# Autodesk Inventor assembly: base_assembly
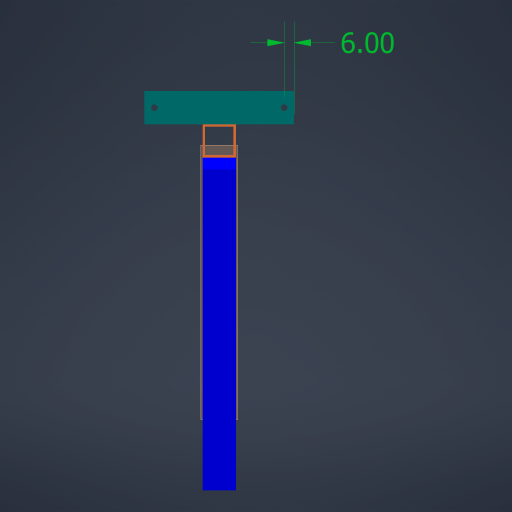
[picture p0: Inventor's stored thumbnail of the model, 512x512]
Saved by Autodesk Inventor 2024 (Build 280153000, 153)
## iProperties
Created: 2023-04-14
Part Number: base_assembly
Document SubType Name: Assembly
Designer: user
Author: user
## Documents named in this file (5)
- D:\Docs\Robot\3d\base\base_assembly.iam
- D:\Docs\Robot\3d\base\main axis.ipt
- D:\Docs\Robot\3d\base\section.ipt
- D:\Docs\Robot\3d\base\shock_absorber_holder_down_150.ipt
- D:\Docs\Robot\3d\base\shock_absorber_holder_down_200.ipt
## Components (8 placed, 4 different names)
1. main axis:1 — Совмещение:1, Совмещение:2, Плоский:1, Плоский:5, Плоский:6, Плоский:8, Совмещение:37, Совмещение:38, Совмещение:41, Совмещение:48, Совмещение:50, Совмещение:52
2. section:1 — Совмещение:1, Совмещение:2, Совмещение:46, Совмещение:49
3. section:3
4. section:4
5. section:5 — Совмещение:45, Совмещение:47, Совмещение:48, Совмещение:49
6. shock_absorber_holder_down_150:1 — Плоский:1, Плоский:8, Совмещение:37, Совмещение:52
7. shock_absorber_holder_down_150:2 — Плоский:5, Плоский:6, Совмещение:50, Совмещение:51
8. shock_absorber_holder_down_200:1 — Совмещение:38, Совмещение:41, Совмещение:51
## Relationships (17: Mate 13, PlanarJoint 4)
- Совмещение:1 [Mate]: main axis:1 ↔ section:1
- Совмещение:2 [Mate] (55 mm): main axis:1 ↔ section:1
- Плоский:1 [PlanarJoint]: main axis:1 ↔ shock_absorber_holder_down_150:1
- Плоский:5 [PlanarJoint]: main axis:1 ↔ shock_absorber_holder_down_150:2
- Плоский:6 [PlanarJoint]: main axis:1 ↔ shock_absorber_holder_down_150:2
- Плоский:8 [PlanarJoint]: main axis:1 ↔ shock_absorber_holder_down_150:1
- Совмещение:37 [Mate]: main axis:1 ↔ shock_absorber_holder_down_150:1
- Совмещение:38 [Mate]: main axis:1 ↔ shock_absorber_holder_down_200:1
- Совмещение:41 [Mate]: main axis:1 ↔ shock_absorber_holder_down_200:1
- Совмещение:45 [Mate]: section:5
- Совмещение:46 [Mate]: section:1
- Совмещение:47 [Mate]: section:5
- Совмещение:48 [Mate]: main axis:1 ↔ section:5
- Совмещение:49 [Mate]: section:1 ↔ section:5
- Совмещение:50 [Mate] (55 mm): main axis:1 ↔ shock_absorber_holder_down_150:2
- Совмещение:51 [Mate] (117 mm): shock_absorber_holder_down_150:2 ↔ shock_absorber_holder_down_200:1
- Совмещение:52 [Mate] (55 mm): main axis:1 ↔ shock_absorber_holder_down_150:1
## Named parameters: hw = 1 mm, up_sh = 40 mm
